# Autodesk Inventor assembly: standing_robot_ver.1
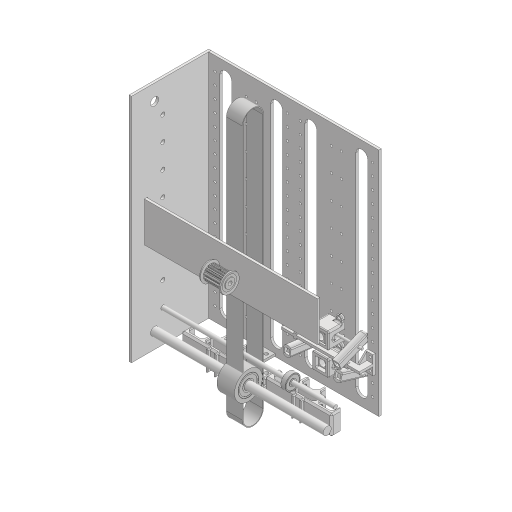
[picture p0: Inventor's stored thumbnail of the model, 512x512]
Saved by Autodesk Inventor 2024 (Build 280153000, 153)
## iProperties
Created: 2023-11-09
Part Number: standing_robot_ver.1
Document SubType Name: Assembly
Designer: moonshot
Author: moonshot
## Documents named in this file (16)
- C:\Users\moonshot\Desktop\ikisawa\ikisawa\experiment8_standing\standing_robot\standing_robot_ver.3.iam
- C:\Users\moonshot\Desktop\ikisawa\ikisawa\experiment8_standing\leg_unit\cover.ver1.ipt
- C:\Users\moonshot\Desktop\ikisawa\ikisawa\experiment8_standing\leg_unit\leg.ipt
- C:\Users\moonshot\Desktop\ikisawa\ikisawa\experiment8_standing\leg_unit\shaft_leg.ipt
- C:\Users\moonshot\Desktop\ikisawa\ikisawa\experiment8_standing\leg_unit\parent_ver.1.ipt
- C:\Users\moonshot\Desktop\ikisawa\ikisawa\experiment8_standing\floor\floor_ver.1.ipt
- C:\Users\moonshot\Desktop\ikisawa\ikisawa\experiment8_standing\belt\ATBT-720T5200-B-P30_info-1-16-16.ipt
- C:\Users\moonshot\Desktop\ikisawa\ikisawa\experiment8_standing\guide\guide_ver.2.ipt
- C:\Users\moonshot\Desktop\ikisawa\ikisawa\experiment8_standing\pulley\AIS2024\TTPS12T5200-A-P5.iam
- C:\Users\moonshot\Desktop\ikisawa\ikisawa\experiment8_standing\adapter\adapter_repulsive_force_ver.3.ipt
- C:\Users\moonshot\Desktop\ikisawa\ikisawa\experiment8_standing\wall\wall_ver.1.ipt
- C:\Users\moonshot\Desktop\ikisawa\ikisawa\experiment8_standing\bearing\C-SE635ZZ.ipt
- C:\Users\moonshot\Desktop\ikisawa\ikisawa\experiment8_standing\bearing\shaft_bearing\shaft_bearing.ipt
- C:\Users\moonshot\Desktop\ikisawa\ikisawa\experiment8_standing\stage\stage_ver.1.ipt
- C:\Users\moonshot\Desktop\ikisawa\ikisawa\experiment8_standing\idler\AIS2024\C-AFBD22-35W.iam
- C:\Users\moonshot\Desktop\ikisawa\ikisawa\experiment8_standing\bearing\shaft_bearing\shaft_idler_ver.1.ipt
## Components (22 placed, 15 different names)
1. cover.ver1:1 — フラッシュ:1, スライダ:1, メイト:8, メイト:9, メイト:10, メイト:36
2. leg:1 — メイト:2, メイト:5
3. leg:2 — メイト:3, メイト:4
4. shaft_leg:1 — メイト:1, フラッシュ:2, メイト:2, メイト:3
5. parent_ver.1:1 — フラッシュ:1, スライダ:1, メイト:1, フラッシュ:2, メイト:41
6. floor_ver.1:1 — フラッシュ:3, フラッシュ:4, フラッシュ:5, メイト:8, メイト:9, メイト:10, メイト:16, メイト:17, メイト:18, メイト:4, メイト:5, メイト:15, メイト:14, メイト:19, メイト:20, メイト:21, メイト:40, フラッシュ:11, フラッシュ:12
7. ATBT-720T5200-B-P30_info-1-16-16:1 — メイト:6, フラッシュ:6, メイト:32, メイト:33, メイト:34, メイト:35
8. cover.ver1:2 — メイト:16, メイト:17, メイト:18
9. leg:3 — メイト:15
10. leg:4 — メイト:14
11. shaft_leg:2
12. parent_ver.1:2
13. guide_ver.2:1 — メイト:19, メイト:20, メイト:21
14. TTPS12T5200-A-P5:1 [sub-assembly] — メイト:29, フラッシュ:9, メイト:50
15. adapter_repulsive_force_ver.3:1 — メイト:30, メイト:31, メイト:32, メイト:33, メイト:34, メイト:36
16. adapter_repulsive_force_ver.3:2 — メイト:30, メイト:31, メイト:35
17. wall_ver.1:2 — メイト:40, フラッシュ:11, フラッシュ:12, フラッシュ:13, メイト:46, フラッシュ:14, メイト:48, メイト:51
18. C-SE635ZZ:1 — メイト:41, メイト:43
19. shaft_bearing:1 — フラッシュ:13, メイト:43, メイト:46
20. stage_ver.1:1 — メイト:44, メイト:45, メイト:50, メイト:51
21. C-AFBD22-35W:1 [sub-assembly] — メイト:47, メイト:49
22. shaft_idler_ver.1:1 — フラッシュ:14, メイト:48, メイト:49
## Relationships (54: Mate 39, Flush 13, TranslationJoint 2)
- フラッシュ:1 [Flush]: cover.ver1:1 ↔ parent_ver.1:1
- スライダ:1 [TranslationJoint]: cover.ver1:1 ↔ parent_ver.1:1
- メイト:1 [Mate]: shaft_leg:1 ↔ parent_ver.1:1
- フラッシュ:2 [Flush]: shaft_leg:1 ↔ parent_ver.1:1
- メイト:2 [Mate]: leg:1 ↔ shaft_leg:1
- メイト:3 [Mate]: leg:2 ↔ shaft_leg:1
- メイト:4 [Mate] (2.5 mm): leg:2 ↔ floor_ver.1:1
- メイト:5 [Mate] (2.5 mm): leg:1 ↔ floor_ver.1:1
- フラッシュ:3 [Flush]: floor_ver.1:1
- フラッシュ:4 [Flush]: floor_ver.1:1
- フラッシュ:5 [Flush]: floor_ver.1:1
- メイト:6 [Mate]: ATBT-720T5200-B-P30_info-1-16-16:1
- フラッシュ:6 [Flush]: ATBT-720T5200-B-P30_info-1-16-16:1
- メイト:8 [Mate]: cover.ver1:1 ↔ floor_ver.1:1
- メイト:9 [Mate]: cover.ver1:1 ↔ floor_ver.1:1
- メイト:10 [Mate]: cover.ver1:1 ↔ floor_ver.1:1
- [Flush]: cover.ver1:2 ↔ parent_ver.1:2
- [TranslationJoint]: cover.ver1:2 ↔ parent_ver.1:2
- [Mate]: shaft_leg:2 ↔ parent_ver.1:2
- [Flush]: shaft_leg:2 ↔ parent_ver.1:2
- [Mate]: leg:3 ↔ shaft_leg:2
- [Mate]: leg:4 ↔ shaft_leg:2
- メイト:14 [Mate] (2.5 mm): floor_ver.1:1 ↔ leg:4
- メイト:15 [Mate] (2.5 mm): floor_ver.1:1 ↔ leg:3
- メイト:16 [Mate]: floor_ver.1:1 ↔ cover.ver1:2
- メイト:17 [Mate]: floor_ver.1:1 ↔ cover.ver1:2
- メイト:18 [Mate]: floor_ver.1:1 ↔ cover.ver1:2
- メイト:19 [Mate]: floor_ver.1:1 ↔ guide_ver.2:1
- メイト:20 [Mate]: floor_ver.1:1 ↔ guide_ver.2:1
- メイト:21 [Mate]: floor_ver.1:1 ↔ guide_ver.2:1
- メイト:29 [Mate]: TTPS12T5200-A-P5:1
- フラッシュ:9 [Flush]: TTPS12T5200-A-P5:1
- メイト:50 [Mate] (13 mm): TTPS12T5200-A-P5:1 ↔ stage_ver.1:1
- メイト:30 [Mate]: adapter_repulsive_force_ver.3:1 ↔ adapter_repulsive_force_ver.3:2
- メイト:31 [Mate]: adapter_repulsive_force_ver.3:1 ↔ adapter_repulsive_force_ver.3:2
- メイト:32 [Mate]: ATBT-720T5200-B-P30_info-1-16-16:1 ↔ adapter_repulsive_force_ver.3:1
- メイト:33 [Mate]: ATBT-720T5200-B-P30_info-1-16-16:1 ↔ adapter_repulsive_force_ver.3:1
- メイト:34 [Mate]: ATBT-720T5200-B-P30_info-1-16-16:1 ↔ adapter_repulsive_force_ver.3:1
- メイト:35 [Mate]: ATBT-720T5200-B-P30_info-1-16-16:1 ↔ adapter_repulsive_force_ver.3:2
- メイト:36 [Mate] (1 mm): cover.ver1:1 ↔ adapter_repulsive_force_ver.3:1
- メイト:40 [Mate]: floor_ver.1:1 ↔ wall_ver.1:2
- フラッシュ:11 [Flush]: floor_ver.1:1 ↔ wall_ver.1:2
- フラッシュ:12 [Flush]: floor_ver.1:1 ↔ wall_ver.1:2
- メイト:41 [Mate]: parent_ver.1:1 ↔ C-SE635ZZ:1
- フラッシュ:13 [Flush]: wall_ver.1:2 ↔ shaft_bearing:1
- メイト:43 [Mate]: C-SE635ZZ:1 ↔ shaft_bearing:1
- メイト:44 [Mate]: stage_ver.1:1
- メイト:45 [Mate]: stage_ver.1:1
- メイト:46 [Mate]: wall_ver.1:2 ↔ shaft_bearing:1
- メイト:47 [Mate]: C-AFBD22-35W:1
- フラッシュ:14 [Flush]: wall_ver.1:2 ↔ shaft_idler_ver.1:1
- メイト:48 [Mate]: wall_ver.1:2 ↔ shaft_idler_ver.1:1
- メイト:49 [Mate]: C-AFBD22-35W:1 ↔ shaft_idler_ver.1:1
- メイト:51 [Mate] (20 mm): wall_ver.1:2 ↔ stage_ver.1:1
## Named parameters: d21_d1 = 0 mm, d22_d2 = 0 mm, d23_d3 = 2 mm, d24_d4 = -2.2469 mm, d25_d5 = -3 mm, d26_d6 = 0 mm, d27_d7 = 0 mm, d28_d8 = 0 mm, d29_d9 = 0 mm, d30_d10 = 2.5 mm, d31_d11 = 2.5 mm
